# Autodesk Inventor assembly: New robot Kicker
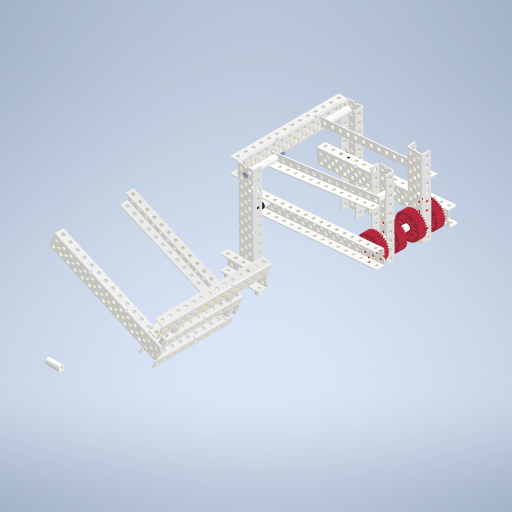
[picture p0: Inventor's stored thumbnail of the model, 512x512]
Saved by Autodesk Inventor 2023 (Build 270158000, 158)
## iProperties
Created: 2023-12-06
Part Number: New robot Kicker
Document SubType Name: Assembly
Designer: Robodox
Author: Robodox
## Documents named in this file (20)
- C:\Users\Robodox\Documents\GitHub\2024-599Z\Cad\New robot Kicker.iam
- C:\Users\Robodox\Documents\GitHub\2024-599Z\Cad\VEX-CAD-Inventor-1.4.0\Structure\C Channel\Aluminum 1x2x1\Alu C 1x2x1x5.ipt
- C:\Users\Robodox\Documents\GitHub\2024-599Z\Cad\VEX-CAD-Inventor-1.4.0\Motion\Spacers\Spacer Nylon .313 OD\NSpacer .313 OD x .250.ipt
- C:\Users\Robodox\Documents\GitHub\2024-599Z\Cad\VEX-CAD-Inventor-1.4.0\Motion\Spacers\Spacer Nylon .313 OD.ipt
- C:\Users\Robodox\Documents\GitHub\2024-599Z\Cad\VEX-CAD-Inventor-1.4.0\Structure\C Channel\Aluminum 1x2x1\Alu C 1x2x1x12.ipt
- C:\Users\Robodox\Documents\GitHub\2024-599Z\Cad\VEX-CAD-Inventor-1.4.0\Motion\Spacers\Spacer Nylon .313 OD\NSpacer .313 OD x .125.ipt
- C:\Users\Robodox\Documents\GitHub\2024-599Z\Cad\VEX-CAD-Inventor-1.4.0\Structure\C Channel\Aluminum 1x2x1\Alu C 1x2x1x14.ipt
- C:\Users\Robodox\Documents\GitHub\2024-599Z\Cad\VEX-CAD-Inventor-1.4.0\Structure\C Channel\Aluminum 1x2x1\Alu C 1x2x1x17.ipt
- C:\Users\Robodox\Documents\GitHub\2024-599Z\Cad\VEX-CAD-Inventor-1.4.0\Motion\Shaft HS\HS Spacer\HSpacer .5000.ipt
- C:\Users\Robodox\Documents\GitHub\2024-599Z\Cad\VEX-CAD-Inventor-1.4.0\Motion\Shaft HS\HS Spacer.ipt
- C:\Users\Robodox\Documents\GitHub\2024-599Z\Cad\VEX-CAD-Inventor-1.4.0\Structure\C Channel\Aluminum 1x2x1\Alu C 1x2x1x10.ipt
- C:\Users\Robodox\Documents\GitHub\2024-599Z\Cad\VEX-CAD-Inventor-1.4.0\Motion\Gears\HS Gear\HS 36T Gear, No Insert.iam
- C:\Users\Robodox\Documents\GitHub\2024-599Z\Cad\VEX-CAD-Inventor-1.4.0\Motion\Gears\HS Gear.iam
- C:\Users\Robodox\Documents\GitHub\2024-599Z\Cad\VEX-CAD-Inventor-1.4.0\Motion\Gears\HS Gear\HS 36T Gear, Square.iam
- C:\Users\Robodox\Documents\GitHub\2024-599Z\Cad\VEX-CAD-Inventor-1.4.0\Motion\Spacers\Spacer Nylon .313 OD\NSpacer .313 OD x .500.ipt
- C:\Users\Robodox\Documents\GitHub\2024-599Z\Cad\VEX-CAD-Inventor-1.4.0\Structure\C Channel\Aluminum 1x3x1 Half\Alu C Half 1x3x1x14.ipt
- C:\Users\Robodox\Documents\GitHub\2024-599Z\Cad\VEX-CAD-Inventor-1.4.0\Structure\Hardware\Screw Steel - Star\SScrew Star Smooth 2.500.ipt
- C:\Users\Robodox\Documents\GitHub\2024-599Z\Cad\VEX-CAD-Inventor-1.4.0\Structure\Hardware\Screw Steel - Star.ipt
- C:\Users\Robodox\Documents\GitHub\2024-599Z\Cad\VEX-CAD-Inventor-1.4.0\Motion\Spacers\Spacer Nylon .313 OD\NSpacer .313 OD x .375.ipt
- C:\Users\Robodox\Documents\GitHub\2024-599Z\Cad\VEX-CAD-Inventor-1.4.0\Structure\C Channel\Aluminum 1x2x1\Alu C 1x2x1x15.ipt
## Components (68 placed, 15 different names)
1. Alu C 1x2x1x5:1
2. NSpacer .313 OD x .250:1
3. NSpacer .313 OD x .250:2
4. Alu C 1x2x1x12:1
5. Alu C 1x2x1x12:2
6. Alu C 1x2x1x5:2
7. NSpacer .313 OD x .250:3
8. NSpacer .313 OD x .250:4
9. NSpacer .313 OD x .125:5
10. NSpacer .313 OD x .125:6
11. NSpacer .313 OD x .125:7
12. NSpacer .313 OD x .125:8
13. Alu C 1x2x1x14:1
14. Alu C 1x2x1x17:1
15. HSpacer .5000:1
16. Alu C 1x2x1x17:2
17. HSpacer .5000:2
18. Alu C 1x2x1x10:1
19. HS 36T Gear, No Insert:1 [sub-assembly]
20. HS 36T Gear, Square:2 [sub-assembly]
21. NSpacer .313 OD x .500:9
22. NSpacer .313 OD x .125:10
23. NSpacer .313 OD x .125:11
24. HS 36T Gear, Square:3 [sub-assembly]
25. NSpacer .313 OD x .500:12
26. Alu C 1x2x1x10:2
27. HS 36T Gear, No Insert:4 [sub-assembly]
28. NSpacer .313 OD x .500:13
29. NSpacer .313 OD x .250:14
30. NSpacer .313 OD x .125:15
31. Alu C Half 1x3x1x14:1
32. SScrew Star Smooth 2.500:1
33. NSpacer .313 OD x .500:16
34. NSpacer .313 OD x .500:17
35. NSpacer .313 OD x .500:18
36. NSpacer .313 OD x .375:19
37. NSpacer .313 OD x .500:20
38. NSpacer .313 OD x .375:21
39. NSpacer .313 OD x .500:22
40. NSpacer .313 OD x .500:23
41. NSpacer .313 OD x .500:24
42. Alu C Half 1x3x1x14:2
43. NSpacer .313 OD x .125:25
44. NSpacer .313 OD x .500:26
45. NSpacer .313 OD x .375:27
46. Alu C 1x2x1x10:3
47. Alu C 1x2x1x15:1
48. Alu C 1x2x1x15:2
49. NSpacer .313 OD x .500:28
50. NSpacer .313 OD x .375:29
51. NSpacer .313 OD x .500:30
52. NSpacer .313 OD x .375:31
53. NSpacer .313 OD x .500:32
54. NSpacer .313 OD x .375:33
55. NSpacer .313 OD x .500:34
56. NSpacer .313 OD x .375:35
57. NSpacer .313 OD x .500:36
58. NSpacer .313 OD x .375:37
59. NSpacer .313 OD x .500:38
60. Alu C 1x2x1x10:4
61. NSpacer .313 OD x .500:39
62. NSpacer .313 OD x .500:40
63. NSpacer .313 OD x .500:41
64. Alu C 1x2x1x14:2
65. NSpacer .313 OD x .500:42
66. NSpacer .313 OD x .375:43
67. NSpacer .313 OD x .500:44
68. NSpacer .313 OD x .375:45
## Relationships (77: Insert 77)
- [Insert]: Alu C 1x2x1x5:1 ↔ NSpacer .313 OD x .250:2
- [Insert]: Alu C 1x2x1x5:2 ↔ NSpacer .313 OD x .250:3
- [Insert]: Alu C 1x2x1x5:2 ↔ NSpacer .313 OD x .250:4
- [Insert]: Alu C 1x2x1x5:2 ↔ NSpacer .313 OD x .125:5
- [Insert]: Alu C 1x2x1x5:2 ↔ NSpacer .313 OD x .125:6
- [Insert]: Alu C 1x2x1x5:1 ↔ NSpacer .313 OD x .125:8
- [Insert]: Alu C 1x2x1x5:1 ↔ NSpacer .313 OD x .125:7
- [Insert]: Alu C 1x2x1x12:2 ↔ NSpacer .313 OD x .125:8
- [Insert]: Alu C 1x2x1x12:2 ↔ NSpacer .313 OD x .125:7
- [Insert]: Alu C 1x2x1x12:1 ↔ NSpacer .313 OD x .125:6
- [Insert]: Alu C 1x2x1x12:1 ↔ NSpacer .313 OD x .125:5
- [Insert]: Alu C 1x2x1x12:1 ↔ Alu C 1x2x1x14:1
- [Insert]: Alu C 1x2x1x12:2 ↔ Alu C 1x2x1x14:1
- [Insert]: Alu C 1x2x1x12:2 ↔ Alu C 1x2x1x14:1
- [Insert]: Alu C 1x2x1x12:1 ↔ Alu C 1x2x1x14:1
- [Insert]: Alu C 1x2x1x17:1 ↔ HS 36T Gear, Square:2
- [Insert]: Alu C 1x2x1x17:1 ↔ HS 36T Gear, Square:2
- [Insert]: HS 36T Gear, Square:2 ↔ NSpacer .313 OD x .500:9
- [Insert]: NSpacer .313 OD x .500:9 ↔ NSpacer .313 OD x .125:11
- [Insert]: Alu C 1x2x1x10:1 ↔ NSpacer .313 OD x .125:11
- [Insert]: Alu C 1x2x1x17:2 ↔ HS 36T Gear, Square:3
- [Insert]: Alu C 1x2x1x17:2 ↔ HS 36T Gear, Square:3
- [Insert]: HS 36T Gear, Square:3 ↔ NSpacer .313 OD x .500:12
- [Insert]: NSpacer .313 OD x .125:10 ↔ NSpacer .313 OD x .500:12
- [Insert]: NSpacer .313 OD x .125:10 ↔ Alu C 1x2x1x10:2
- [Insert]: Alu C 1x2x1x10:1 ↔ HS 36T Gear, No Insert:4
- [Insert]: HS 36T Gear, No Insert:1 ↔ Alu C 1x2x1x10:2
- [Insert]: HS 36T Gear, No Insert:4 ↔ NSpacer .313 OD x .500:13
- [Insert]: HS 36T Gear, No Insert:1 ↔ NSpacer .313 OD x .250:14
- [Insert]: Alu C 1x2x1x10:1 ↔ NSpacer .313 OD x .125:15
- [Insert]: Alu C 1x2x1x12:1 ↔ SScrew Star Smooth 2.500:1
- [Insert]: Alu C 1x2x1x12:1 ↔ NSpacer .313 OD x .500:16
- [Insert]: NSpacer .313 OD x .500:16 ↔ NSpacer .313 OD x .500:17
- [Insert]: NSpacer .313 OD x .500:18 ↔ NSpacer .313 OD x .375:19
- [Insert]: Alu C Half 1x3x1x14:1 ↔ NSpacer .313 OD x .375:19
- [Insert]: NSpacer .313 OD x .125:15 ↔ NSpacer .313 OD x .500:20
- [Insert]: Alu C Half 1x3x1x14:1 ↔ NSpacer .313 OD x .500:20
- [Insert]: NSpacer .313 OD x .500:17 ↔ NSpacer .313 OD x .500:18
- [Insert]: Alu C 1x2x1x17:1 ↔ NSpacer .313 OD x .375:21
- [Insert]: HSpacer .5000:1 ↔ NSpacer .313 OD x .375:21
- [Insert]: NSpacer .313 OD x .500:22 ↔ NSpacer .313 OD x .500:23
- [Insert]: NSpacer .313 OD x .500:23 ↔ NSpacer .313 OD x .500:24
- [Insert]: NSpacer .313 OD x .500:22 ↔ Alu C Half 1x3x1x14:2
- [Insert]: NSpacer .313 OD x .125:25 ↔ NSpacer .313 OD x .500:26
- [Insert]: Alu C Half 1x3x1x14:2 ↔ NSpacer .313 OD x .500:26
- [Insert]: Alu C 1x2x1x10:2 ↔ NSpacer .313 OD x .125:25
- [Insert]: HSpacer .5000:2 ↔ NSpacer .313 OD x .375:27
- [Insert]: Alu C 1x2x1x17:2 ↔ NSpacer .313 OD x .375:27
- [Insert]: NSpacer .313 OD x .500:13 ↔ NSpacer .313 OD x .250:14
- [Insert]: Alu C 1x2x1x5:1 ↔ NSpacer .313 OD x .250:1
- [Insert]: Alu C 1x2x1x10:3 ↔ Alu C 1x2x1x15:1
- [Insert]: Alu C 1x2x1x10:3 ↔ Alu C 1x2x1x15:1
- [Insert]: Alu C 1x2x1x10:3 ↔ Alu C 1x2x1x15:2
- [Insert]: Alu C 1x2x1x10:3 ↔ Alu C 1x2x1x15:2
- [Insert]: NSpacer .313 OD x .500:28 ↔ NSpacer .313 OD x .375:29
- [Insert]: NSpacer .313 OD x .500:30 ↔ NSpacer .313 OD x .375:31
- [Insert]: NSpacer .313 OD x .500:32 ↔ NSpacer .313 OD x .375:33
- [Insert]: NSpacer .313 OD x .500:34 ↔ NSpacer .313 OD x .375:35
- [Insert]: NSpacer .313 OD x .500:36 ↔ NSpacer .313 OD x .375:37
- [Insert]: Alu C 1x2x1x15:1 ↔ NSpacer .313 OD x .500:28
- [Insert]: Alu C 1x2x1x15:1 ↔ NSpacer .313 OD x .500:30
- [Insert]: Alu C 1x2x1x15:2 ↔ NSpacer .313 OD x .500:32
- [Insert]: Alu C 1x2x1x15:2 ↔ NSpacer .313 OD x .500:34
- [Insert]: Alu C 1x2x1x15:1 ↔ NSpacer .313 OD x .500:38
- [Insert]: NSpacer .313 OD x .500:38 ↔ Alu C 1x2x1x10:4
- [Insert]: Alu C 1x2x1x15:1 ↔ NSpacer .313 OD x .500:39
- [Insert]: Alu C 1x2x1x15:2 ↔ NSpacer .313 OD x .500:40
- [Insert]: Alu C 1x2x1x15:2 ↔ NSpacer .313 OD x .500:41
- [Insert]: Alu C 1x2x1x10:4 ↔ NSpacer .313 OD x .500:41
- [Insert]: Alu C 1x2x1x10:4 ↔ NSpacer .313 OD x .500:40
- [Insert]: Alu C 1x2x1x10:4 ↔ NSpacer .313 OD x .500:39
- [Insert]: NSpacer .313 OD x .500:42 ↔ NSpacer .313 OD x .375:43
- [Insert]: Alu C 1x2x1x14:2 ↔ NSpacer .313 OD x .375:43
- [Insert]: NSpacer .313 OD x .500:44 ↔ NSpacer .313 OD x .375:45
- [Insert]: Alu C 1x2x1x14:2 ↔ NSpacer .313 OD x .375:45
- [Insert]: Alu C 1x2x1x10:4 ↔ NSpacer .313 OD x .500:44
- [Insert]: Alu C 1x2x1x10:4 ↔ NSpacer .313 OD x .500:42
## Named parameters: d949_d935_d931 = 0 mm, d951_d935_d931 = 0 mm, d932_d931 = 0 mm, d933_d931 = 0 mm, d934_d931 = 0 mm, d935_d931 = 0 mm, d851_d823 = 0 mm, d852_d825 = 0 mm, d853_d826 = 0 mm, d854_d827 = 0 mm, d855_d828 = 0 mm, d856_d829 = 0 mm, d857_d832 = 0 mm, d858_d833 = 0 mm, d859_d834_d823 = 0 mm, d860_d836_d829 = 0 mm, d861_d838 = 0 mm, d862_d839_d827 = 0 mm, d863_d840 = 0 mm, d864_d841 = 0 mm, d865_d843 = 0 mm, d866_d844 = 0 mm, d867_d845 = 0 mm, d868_d794 = 0 mm, d869_d795 = 0 mm, d870_d796 = 0 mm, d871_d797 = 0 mm, d872_d798 = 0 mm, d873_d799 = 0 mm, d874_d800 = 0 mm, d875_d802 = 0 mm, d876_d803 = 0 mm, d877_d804 = 0 mm, d878_d805 = 0 mm, d879_d816 = 0 mm, d880_d818 = 0 mm, d881_d821 = 0 mm, d882_d822 = 0 mm, d883_d792 = 0 mm, d884_d793 = 0 mm, d885_d712 = 0 mm, d886_d740_d730_d711 = 0 mm, d887_d741_d731_d712 = 0 mm, d888_d749 = 0 mm, d889_d750 = 0 mm, d890_d751 = 0 mm, d891_d752 = 0 mm, d892_d753 = 0 mm, d893_d754 = 0 mm, d894_d755 = 0 mm, d895_d756 = 0 mm, d896_d757 = 0 mm, d897_d758 = 0 mm, d898_d759 = 0 mm, d899_d760 = 0 mm
